# Autodesk Inventor assembly: tower_V2
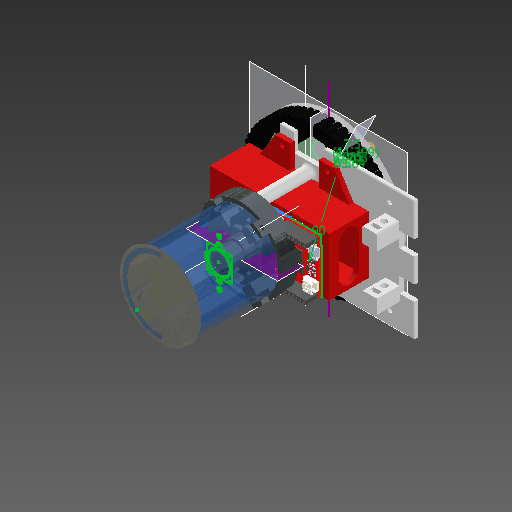
[picture p0: Inventor's stored thumbnail of the model, 512x512]
Saved by Autodesk Inventor 2023 (Build 270158000, 158)
## iProperties
Created: 2025-08-06
Part Number: tower_V2
Document SubType Name: Assembly
Designer: daa
Author: daa
## Documents named in this file (6)
- C:\Users\daa\Documents\DASH_V2\tower_V2.iam
- C:\Users\daa\Documents\DASH_V2\tssop.iam
- C:\Users\daa\Documents\DASH_V2\Dribler_v2\kreplenie_dribler_V4.ipt
- C:\Users\daa\Documents\DASH_V2\akb_mount.ipt
- C:\Users\daa\Documents\DASH_V2\openmv_cennt.iam
- C:\Users\daa\Documents\DASH_V2\rack_25.ipt
## Components (8 placed, 5 different names)
1. tssop:1 [sub-assembly] — Совмещение:1, Совмещение:5, Совмещение:6, Совмещение:7, Совмещение:8
2. kreplenie_dribler_V4:1 — Совмещение:1, Совмещение:2, Совмещение:3, С поворотом:1, Совмещение:4
3. akb_mount:1 — Совмещение:2, Совмещение:3
4. openmv_cennt:1 [sub-assembly] — С поворотом:1, Совмещение:4
5. rack_25:1 — Совмещение:7
6. rack_25:2 — Совмещение:8
7. rack_25:3 — Совмещение:6
8. rack_25:4 — Совмещение:5
## Relationships (9: Mate 8, RevoluteJoint 1)
- Совмещение:1 [Mate]: tssop:1 ↔ kreplenie_dribler_V4:1
- Совмещение:2 [Mate]: kreplenie_dribler_V4:1 ↔ akb_mount:1
- Совмещение:3 [Mate]: kreplenie_dribler_V4:1 ↔ akb_mount:1
- С поворотом:1 [RevoluteJoint]: kreplenie_dribler_V4:1 ↔ openmv_cennt:1
- Совмещение:4 [Mate]: kreplenie_dribler_V4:1 ↔ openmv_cennt:1
- Совмещение:5 [Mate]: tssop:1 ↔ rack_25:4
- Совмещение:6 [Mate]: tssop:1 ↔ rack_25:3
- Совмещение:7 [Mate]: tssop:1 ↔ rack_25:1
- Совмещение:8 [Mate]: tssop:1 ↔ rack_25:2
